# Autodesk Inventor assembly: PhenolicCap
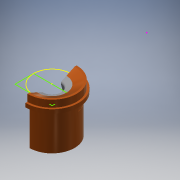
[picture p0: Inventor's stored thumbnail of the model, 180x180]
Saved by Autodesk Inventor 2017 (Build 210142000, 142)
## iProperties
Created: 2016-10-18
Part Number: PhenolicCap
Document SubType Name: Assembly
Designer: hyhe
Author: hyhe
## Documents named in this file (4)
- C:\Users\hyhe\Desktop\PhenolicCap.iam
- C:\Users\hyhe\Downloads\part 1 phenolic sketch.ipt
- C:\Users\hyhe\Downloads\Graphite Master Sketch.ipt
- C:\Users\hyhe\Downloads\part 2 cap of Phenolic Master Sketch.ipt
## Components (3 placed, 3 different names)
1. part 1 phenolic sketch:1 — Mate:1, Mate:2
2. Graphite Master Sketch:1 — Mate:1
3. part 2 cap of Phenolic Master Sketch:1 — Mate:2
## Relationships (2: Mate 2)
- Mate:1: part 1 phenolic sketch:1 ↔ Graphite Master Sketch:1
- Mate:2: part 1 phenolic sketch:1 ↔ part 2 cap of Phenolic Master Sketch:1
